# Autodesk Inventor assembly: chair
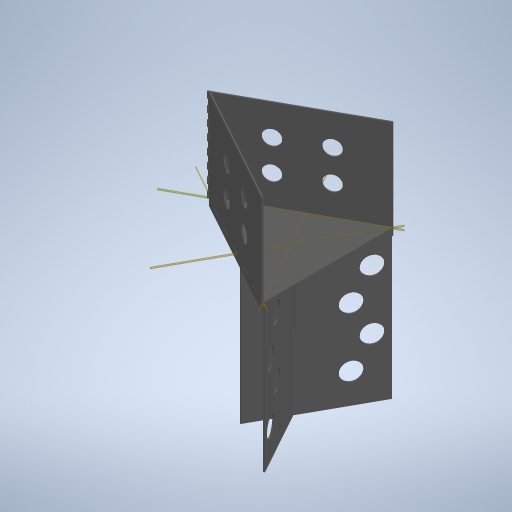
[picture p0: Inventor's stored thumbnail of the model, 512x512]
Saved by Autodesk Inventor 2023 (Build 270158000, 158)
## iProperties
Created: 2023-09-18
Part Number: chair
Document SubType Name: Assembly
Designer: Nate
Mass: 447.241 g
Surface Area: 13853.3 cm^2
Volume: 3149.59 cm^3
Density: 0.142 g/cm^3
Author: Nate
## Documents named in this file (12)
- C:\Users\Nate\Desktop\foam core chair\chair.iam
- C:\Users\Nate\Desktop\foam core chair\chair seat.ipt
- C:\Users\Nate\Desktop\foam core chair\left back.ipt
- C:\Users\Nate\Desktop\foam core chair\right back.ipt
- C:\Users\Nate\Desktop\foam core chair\leg 1.ipt
- C:\Users\Nate\Desktop\foam core chair\leg 2.ipt
- C:\Users\Nate\Desktop\foam core chair\chair\AIP\FEA\egmvpmxds.fins
- C:\Users\Nate\Desktop\foam core chair\chair\AIP\FEA\egmvpmxds.fsat
- C:\Users\Nate\Desktop\foam core chair\chair\AIP\FEA\egmvpmxds.ftes
- C:\Users\Nate\Desktop\foam core chair\chair\AIP\FEA\egmvpmxds.fwiz
- C:\Users\Nate\Desktop\foam core chair\chair\AIP\FEA\egmvpmxq8.fmsh
- C:\Users\Nate\Desktop\foam core chair\chair\AIP\FEA\egmvpmxq9.fres
## Components (5 placed, 5 different names)
1. chair seat:1 — Flush:1, Flush:3, Flush:4, Flush:5, Flush:7, Flush:10, Flush:11
2. left back:1 — Flush:2, Flush:3
3. right back:1 — Flush:5, Flush:6
4. leg 1:1 — Flush:8, Flush:9
5. leg 2:1 — Flush:11, Flush:12
## Relationships (12: Flush 12)
- Flush:1: chair seat:1
- Flush:2: left back:1
- Flush:3: chair seat:1 ↔ left back:1
- Flush:4: chair seat:1
- Flush:5: chair seat:1 ↔ right back:1
- Flush:6: right back:1
- Flush:7: chair seat:1
- Flush:8: leg 1:1
- Flush:9: leg 1:1
- Flush:10: chair seat:1
- Flush:11: chair seat:1 ↔ leg 2:1
- Flush:12: leg 2:1
## Named parameters: sa_0 = 200000, sa_1 = 50000, sa_2 = 50000
note: some values were not read from the file. Shown as the stored number, unit unknown: "sa_0", "sa_1", "sa_2".
